# Autodesk Inventor assembly: Julie
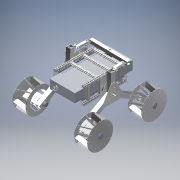
[picture p0: Inventor's stored thumbnail of the model, 180x180]
Saved by Autodesk Inventor 2019 (Build 230136000, 136)
## iProperties
Created: 2018-10-29
Part Number: Julie
Document SubType Name: Assembly
Designer: Adhik
Mass: 18590.5 g
Surface Area: 55652.5 cm^2
Volume: 6942.59 cm^3
Density: 2.67774 g/cm^3
Author: Adhik
## Documents named in this file (21)
- C:\Users\mcgowc2\Desktop\Rock Raiders\Chassis_Final\Julie.iam
- C:\Users\mcgowc2\Desktop\Rock Raiders\Chassis_Final\Baseplate.ipt
- C:\Users\mcgowc2\Desktop\Rock Raiders\Chassis_Final\8020 20 inch lower.ipt
- C:\Users\mcgowc2\Desktop\Rock Raiders\Chassis_Final\8020 12 inch.ipt
- C:\Users\mcgowc2\Desktop\Rock Raiders\Chassis_Final\8020 6 inch.ipt
- C:\Users\mcgowc2\Desktop\Rock Raiders\Chassis_Final\8020 20 inch upper.ipt
- C:\Users\mcgowc2\Desktop\Rock Raiders\Chassis_Final\Lateral Plate.ipt
- C:\Users\mcgowc2\Desktop\Rock Raiders\Chassis_Final\Main Joint.ipt
- C:\Users\mcgowc2\Desktop\Rock Raiders\Chassis_Final\Main Axle.ipt
- C:\Users\mcgowc2\Desktop\Rock Raiders\Chassis_Final\Drive.iam
- C:\Users\mcgowc2\Desktop\Rock Raiders\Chassis_Final\Ball Joint.ipt
- C:\Users\mcgowc2\Desktop\Rock Raiders\Chassis_Final\Arm 8 inch.ipt
- C:\Users\mcgowc2\Desktop\Rock Raiders\Chassis_Final\Coupler.ipt
- C:\Users\mcgowc2\Desktop\Rock Raiders\Chassis_Final\Crossbeam.ipt
- C:\Users\mcgowc2\Desktop\Rock Raiders\Chassis_Final\Arm Bearing.ipt
- C:\Users\mcgowc2\Desktop\Rock Raiders\Chassis_Final\Mounted Bearing.ipt
- C:\Users\mcgowc2\Desktop\Rock Raiders\Chassis_Final\Side Panel.ipt
- C:\Users\mcgowc2\Desktop\Rock Raiders\Chassis_Final\Electrical_Components\RPI_Rock_Raiders_Enclosure_Body.ipt
- C:\Users\mcgowc2\Desktop\Rock Raiders\Chassis_Final\Electrical_Components\RPI_Rock_Raiders_Enclosure_Lid.ipt
- C:\Users\mcgowc2\Desktop\Rock Raiders\Chassis_Final\Electrical_Components\T_Aluminum_No_Slot.ipt
- C:\Users\mcgowc2\Desktop\Rock Raiders\Chassis_Final\Electrical_Components\T_Aluminum_Slot.ipt
## Components (47 placed, 20 different names)
1. Baseplate:1 — Mate:1, Mate:2, Flush:1, Flush:2, Flush:3, Flush:4, Mate:3, Mate:4
2. 8020 20 inch lower:1 — Mate:1, Flush:1, Flush:2, Mate:5, Mate:6, Mate:7, Mate:8, Mate:9, Mate:10, Flush:7, Flush:8, Mate:13, Mate:14, Mate:17, Mate:19, Flush:9, Flush:10, Mate:23, Mate:24, Mate:29, Flush:16, Flush:24, Mate:87
3. 8020 20 inch lower:2 — Mate:2, Flush:3, Flush:4, Mate:11, Mate:12, Flush:5, Flush:6, Mate:15, Mate:16, Mate:18, Mate:20, Flush:11, Flush:12, Mate:21, Mate:22, Mate:30, Flush:17, Flush:26
4. 8020 12 inch:1 — Mate:3, Mate:5, Mate:7
5. 8020 12 inch:2 — Mate:4, Mate:6, Mate:8
6. 8020 6 inch:1 — Mate:9, Flush:7, Mate:13, Mate:26, Flush:14, Flush:15
7. 8020 6 inch:2 — Mate:10, Flush:8, Mate:14, Mate:27
8. 8020 6 inch:3 — Mate:11, Flush:6, Mate:15, Flush:13
9. 8020 6 inch:4 — Mate:12, Flush:5, Mate:16, Mate:28, Flush:18
10. 8020 6 inch:5 — Mate:17, Flush:10, Mate:23
11. 8020 6 inch:6 — Mate:19, Flush:9, Mate:24
12. 8020 6 inch:7 — Mate:18, Flush:12, Mate:21, Mate:86
13. 8020 6 inch:8 — Mate:20, Flush:11, Mate:22, Mate:25
14. 8020 20 inch upper:1 — Mate:25, Flush:13, Mate:28, Mate:66, Flush:21, Mate:74, Mate:75, Flush:27, Flush:28, Flush:29
15. 8020 20 inch upper:2 — Mate:26, Flush:14, Mate:27, Mate:31, Mate:32, Flush:19, Flush:20, Mate:33, Mate:34, Mate:72, Mate:73, Flush:22, Flush:23, Flush:25, Flush:34
16. Lateral Plate:1 — Mate:30, Flush:17, Flush:18, Mate:35, Mate:37, Mate:38
17. Lateral Plate:2 — Mate:29, Flush:15, Flush:16, Mate:36, Mate:39, Mate:40
18. 8020 12 inch:3 — Mate:31, Flush:20, Mate:33
19. 8020 12 inch:4 — Mate:32, Flush:19, Mate:34
20. Main Joint:1 — Mate:35, Mate:37, Mate:38, Mate:42, Mate:45
21. Main Joint:2 — Mate:36, Mate:39, Mate:40, Mate:46
22. Main Axle:1 — Mate:41, Mate:42, Mate:43, Mate:44
23. Drive:1 [sub-assembly] — Mate:44, Mate:45, Mate:47, Mate:48, Mate:49
24. Drive:2 [sub-assembly] — Mate:43, Mate:46, Mate:50, Mate:51, Mate:52
25. Arm 8 inch:1 — Mate:47, Mate:48, Mate:49, Mate:53, Angle:1, Mate:55
26. Arm 8 inch:2 — Mate:50, Mate:51, Mate:52, Mate:54, Angle:2, Mate:56
27. Ball Joint:1 — Mate:53, Angle:1, Mate:55, Mate:57
28. Ball Joint:2 — Mate:54, Angle:2, Mate:56, Mate:58
29. Coupler:1 — Mate:57, Mate:64
30. Coupler:2 — Mate:58, Mate:63
31. Crossbeam:1 — Mate:59, Angle:3, Mate:60, Mate:61, Angle:4, Mate:62, Angle:5, Mate:65, Insert:1, Insert:2, Mate:71
32. Ball Joint:3 — Mate:61, Angle:4, Mate:62, Mate:63
33. Ball Joint:4 — Mate:59, Angle:3, Mate:60, Mate:64
34. 8020 12 inch:5 — Mate:66, Flush:21, Mate:67, Mate:68, Mate:69, Mate:71
35. Arm Bearing:1 — Insert:1
36. Arm Bearing:2 — Insert:2, Mate:70
37. Mounted Bearing:1 — Mate:67, Mate:68, Mate:69, Mate:70
38. Side Panel:1 — Mate:72, Flush:22, Flush:23
39. Side Panel:2 — Mate:75, Flush:28, Flush:29
40. Side Panel:3 — Mate:73, Flush:24, Flush:25
41. Side Panel:4 — Mate:74, Flush:26, Flush:27
42. RPI_Rock_Raiders_Enclosure_Body:1 — Mate:76, Mate:77, Angle:6, Mate:78, Mate:79, Mate:82, Mate:83, Mate:84, Mate:85, Flush:30, Flush:31, Flush:32, Flush:33, Mate:87
43. RPI_Rock_Raiders_Enclosure_Lid:1 — Mate:76, Mate:77, Angle:6, Mate:80, Mate:81
44. T_Aluminum_No_Slot:1 — Mate:81, Mate:83, Flush:30
45. T_Aluminum_No_Slot:2 — Mate:80, Mate:85, Flush:31, Mate:86
46. T_Aluminum_Slot:1 — Mate:78, Mate:84, Flush:32
47. T_Aluminum_Slot:2 — Mate:79, Mate:82, Flush:33, Flush:34
## Relationships (129: Mate 87, Flush 34, Angle 6, Insert 2)
- Mate:1: Baseplate:1 ↔ 8020 20 inch lower:1
- Mate:2: Baseplate:1 ↔ 8020 20 inch lower:2
- Flush:1: Baseplate:1 ↔ 8020 20 inch lower:1
- Flush:2: Baseplate:1 ↔ 8020 20 inch lower:1
- Flush:3: Baseplate:1 ↔ 8020 20 inch lower:2
- Flush:4: Baseplate:1 ↔ 8020 20 inch lower:2
- Mate:3: Baseplate:1 ↔ 8020 12 inch:1
- Mate:4: Baseplate:1 ↔ 8020 12 inch:2
- Mate:5: 8020 20 inch lower:1 ↔ 8020 12 inch:1
- Mate:6: 8020 20 inch lower:1 ↔ 8020 12 inch:2
- Mate:7: 8020 20 inch lower:1 ↔ 8020 12 inch:1
- Mate:8: 8020 20 inch lower:1 ↔ 8020 12 inch:2
- Mate:9: 8020 20 inch lower:1 ↔ 8020 6 inch:1
- Mate:10: 8020 20 inch lower:1 ↔ 8020 6 inch:2
- Mate:11: 8020 20 inch lower:2 ↔ 8020 6 inch:3
- Mate:12: 8020 20 inch lower:2 ↔ 8020 6 inch:4
- Flush:5: 8020 20 inch lower:2 ↔ 8020 6 inch:4
- Flush:6: 8020 20 inch lower:2 ↔ 8020 6 inch:3
- Flush:7: 8020 20 inch lower:1 ↔ 8020 6 inch:1
- Flush:8: 8020 20 inch lower:1 ↔ 8020 6 inch:2
- Mate:13: 8020 20 inch lower:1 ↔ 8020 6 inch:1
- Mate:14: 8020 20 inch lower:1 ↔ 8020 6 inch:2
- Mate:15: 8020 20 inch lower:2 ↔ 8020 6 inch:3
- Mate:16: 8020 20 inch lower:2 ↔ 8020 6 inch:4
- Mate:17: 8020 20 inch lower:1 ↔ 8020 6 inch:5
- Mate:18: 8020 20 inch lower:2 ↔ 8020 6 inch:7
- Mate:19: 8020 20 inch lower:1 ↔ 8020 6 inch:6
- Mate:20: 8020 20 inch lower:2 ↔ 8020 6 inch:8
- Flush:9: 8020 20 inch lower:1 ↔ 8020 6 inch:6
- Flush:10: 8020 20 inch lower:1 ↔ 8020 6 inch:5
- Flush:11: 8020 20 inch lower:2 ↔ 8020 6 inch:8
- Flush:12: 8020 20 inch lower:2 ↔ 8020 6 inch:7
- Mate:21: 8020 20 inch lower:2 ↔ 8020 6 inch:7
- Mate:22: 8020 20 inch lower:2 ↔ 8020 6 inch:8
- Mate:23: 8020 20 inch lower:1 ↔ 8020 6 inch:5
- Mate:24: 8020 20 inch lower:1 ↔ 8020 6 inch:6
- Mate:25: 8020 6 inch:8 ↔ 8020 20 inch upper:1
- Flush:13: 8020 6 inch:3 ↔ 8020 20 inch upper:1
- Mate:26: 8020 6 inch:1 ↔ 8020 20 inch upper:2
- Flush:14: 8020 6 inch:1 ↔ 8020 20 inch upper:2
- Mate:27: 8020 6 inch:2 ↔ 8020 20 inch upper:2
- Mate:28: 8020 6 inch:4 ↔ 8020 20 inch upper:1
- Mate:29: 8020 20 inch lower:1 ↔ Lateral Plate:2
- Flush:15: 8020 6 inch:1 ↔ Lateral Plate:2
- Flush:16: 8020 20 inch lower:1 ↔ Lateral Plate:2
- Mate:30: 8020 20 inch lower:2 ↔ Lateral Plate:1
- Flush:17: 8020 20 inch lower:2 ↔ Lateral Plate:1
- Flush:18: 8020 6 inch:4 ↔ Lateral Plate:1
- Mate:31: 8020 20 inch upper:2 ↔ 8020 12 inch:3
- Mate:32: 8020 20 inch upper:2 ↔ 8020 12 inch:4
- Flush:19: 8020 20 inch upper:2 ↔ 8020 12 inch:4
- Flush:20: 8020 20 inch upper:2 ↔ 8020 12 inch:3
- Mate:33: 8020 20 inch upper:2 ↔ 8020 12 inch:3
- Mate:34: 8020 20 inch upper:2 ↔ 8020 12 inch:4
- Mate:35: Lateral Plate:1 ↔ Main Joint:1
- Mate:36: Lateral Plate:2 ↔ Main Joint:2
- Mate:37: Lateral Plate:1 ↔ Main Joint:1
- Mate:38: Lateral Plate:1 ↔ Main Joint:1
- Mate:39: Lateral Plate:2 ↔ Main Joint:2
- Mate:40: Lateral Plate:2 ↔ Main Joint:2
- Mate:41: Main Axle:1
- Mate:42: Main Joint:1 ↔ Main Axle:1
- Mate:43: Main Axle:1 ↔ Drive:2
- Mate:44: Main Axle:1 ↔ Drive:1
- Mate:45: Main Joint:1 ↔ Drive:1
- Mate:46: Main Joint:2 ↔ Drive:2
- Mate:47: Drive:1 ↔ Arm 8 inch:1
- Mate:48: Drive:1 ↔ Arm 8 inch:1
- Mate:49: Drive:1 ↔ Arm 8 inch:1
- Mate:50: Drive:2 ↔ Arm 8 inch:2
- Mate:51: Drive:2 ↔ Arm 8 inch:2
- Mate:52: Drive:2 ↔ Arm 8 inch:2
- Mate:53: Arm 8 inch:1 ↔ Ball Joint:1
- Angle:1 (0 deg): Arm 8 inch:1 ↔ Ball Joint:1
- Mate:54: Arm 8 inch:2 ↔ Ball Joint:2
- Angle:2 (0 deg): Arm 8 inch:2 ↔ Ball Joint:2
- Mate:55 (12.7 mm): Arm 8 inch:1 ↔ Ball Joint:1
- Mate:56 (12.7 mm): Arm 8 inch:2 ↔ Ball Joint:2
- Mate:57: Ball Joint:1 ↔ Coupler:1
- Mate:58: Ball Joint:2 ↔ Coupler:2
- Mate:59: Crossbeam:1 ↔ Ball Joint:4
- Angle:3 (0 deg): Crossbeam:1 ↔ Ball Joint:4
- Mate:60 (19.05 mm): Crossbeam:1 ↔ Ball Joint:4
- Mate:61: Crossbeam:1 ↔ Ball Joint:3
- Angle:4 (0 deg): Crossbeam:1 ↔ Ball Joint:3
- Mate:62 (19.05 mm): Crossbeam:1 ↔ Ball Joint:3
- Mate:63: Coupler:2 ↔ Ball Joint:3
- Mate:64: Coupler:1 ↔ Ball Joint:4
- Angle:5 (0 deg): Crossbeam:1
- Mate:65: Crossbeam:1
- Mate:66: 8020 20 inch upper:1 ↔ 8020 12 inch:5
- Flush:21: 8020 20 inch upper:1 ↔ 8020 12 inch:5
- Insert:1: Crossbeam:1 ↔ Arm Bearing:1
- Insert:2: Crossbeam:1 ↔ Arm Bearing:2
- Mate:67: 8020 12 inch:5 ↔ Mounted Bearing:1
- Mate:68: 8020 12 inch:5 ↔ Mounted Bearing:1
- Mate:69: 8020 12 inch:5 ↔ Mounted Bearing:1
- Mate:70: Arm Bearing:2 ↔ Mounted Bearing:1
- Mate:71 (6.35 mm): Crossbeam:1 ↔ 8020 12 inch:5
- Mate:72: 8020 20 inch upper:2 ↔ Side Panel:1
- Mate:73: 8020 20 inch upper:2 ↔ Side Panel:3
- Mate:74: 8020 20 inch upper:1 ↔ Side Panel:4
- Mate:75: 8020 20 inch upper:1 ↔ Side Panel:2
- Flush:22: 8020 20 inch upper:2 ↔ Side Panel:1
- Flush:23: 8020 20 inch upper:2 ↔ Side Panel:1
- Flush:24: 8020 20 inch lower:1 ↔ Side Panel:3
- Flush:25: 8020 20 inch upper:2 ↔ Side Panel:3
- Flush:26: 8020 20 inch lower:2 ↔ Side Panel:4
- Flush:27: 8020 20 inch upper:1 ↔ Side Panel:4
- Flush:28: 8020 20 inch upper:1 ↔ Side Panel:2
- Flush:29: 8020 20 inch upper:1 ↔ Side Panel:2
- Mate:76: RPI_Rock_Raiders_Enclosure_Body:1 ↔ RPI_Rock_Raiders_Enclosure_Lid:1
- Mate:77: RPI_Rock_Raiders_Enclosure_Body:1 ↔ RPI_Rock_Raiders_Enclosure_Lid:1
- Angle:6 (0 deg): RPI_Rock_Raiders_Enclosure_Body:1 ↔ RPI_Rock_Raiders_Enclosure_Lid:1
- Mate:78: RPI_Rock_Raiders_Enclosure_Body:1 ↔ T_Aluminum_Slot:1
- Mate:79: RPI_Rock_Raiders_Enclosure_Body:1 ↔ T_Aluminum_Slot:2
- Mate:80: RPI_Rock_Raiders_Enclosure_Lid:1 ↔ T_Aluminum_No_Slot:2
- Mate:81: RPI_Rock_Raiders_Enclosure_Lid:1 ↔ T_Aluminum_No_Slot:1
- Mate:82: RPI_Rock_Raiders_Enclosure_Body:1 ↔ T_Aluminum_Slot:2
- Mate:83: RPI_Rock_Raiders_Enclosure_Body:1 ↔ T_Aluminum_No_Slot:1
- Mate:84: RPI_Rock_Raiders_Enclosure_Body:1 ↔ T_Aluminum_Slot:1
- Mate:85: RPI_Rock_Raiders_Enclosure_Body:1 ↔ T_Aluminum_No_Slot:2
- Flush:30 (127 mm): RPI_Rock_Raiders_Enclosure_Body:1 ↔ T_Aluminum_No_Slot:1
- Flush:31 (127 mm): RPI_Rock_Raiders_Enclosure_Body:1 ↔ T_Aluminum_No_Slot:2
- Flush:32 (76.2 mm): RPI_Rock_Raiders_Enclosure_Body:1 ↔ T_Aluminum_Slot:1
- Flush:33 (76.2 mm): RPI_Rock_Raiders_Enclosure_Body:1 ↔ T_Aluminum_Slot:2
- Mate:86 (1.5875 mm): 8020 6 inch:7 ↔ T_Aluminum_No_Slot:2
- Flush:34: 8020 20 inch upper:2 ↔ T_Aluminum_Slot:2
- Mate:87 (25.4 mm): 8020 20 inch lower:1 ↔ RPI_Rock_Raiders_Enclosure_Body:1
